# Autodesk Inventor assembly: Frame
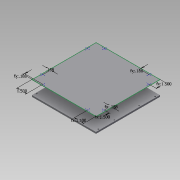
[picture p0: Inventor's stored thumbnail of the model, 180x180]
Saved by Autodesk Inventor 2,016 (Build 200138000, 138)
## iProperties
Created: 2017-05-15
Part Number: Frame
Document SubType Name: Assembly
Designer: 31745
Author: 31745
## Documents named in this file (4)
- H:\Projects\Printer #2\IAM\Frame.iam
- H:\Projects\Printer #2\IPT\Machined Parts\Base.ipt
- H:\Projects\Printer #2\IPT\Machined Parts\Print Bed.ipt
- H:\Projects\Printer #2\IPT\Machined Parts\XY Carriage.ipt
## Components (3 placed, 3 different names)
1. Base:1 — Mate:1, Mate:2, Flush:1, Flush:2
2. Print Bed:1 — Mate:1, Mate:2
3. XY Carriage:1 — Flush:1, Flush:2
## Relationships (4: Mate 2, Flush 2)
- Mate:1: Base:1 ↔ Print Bed:1
- Mate:2: Base:1 ↔ Print Bed:1
- Flush:1: Base:1 ↔ XY Carriage:1
- Flush:2: Base:1 ↔ XY Carriage:1
